# Autodesk Inventor assembly: CKK_145_NN_1_1800_mm_MF01_03_34_309_033
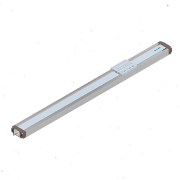
[picture p0: Inventor's stored thumbnail of the model, 180x180]
Saved by Autodesk Inventor 2021 (Build 250183000, 183)
## iProperties
Created: 2021-03-29
Part Number: CKK_145_NN_1_1800_mm_MF01_03_34_309_033
Document SubType Name: Assembly
Designer: Work
Sending System: CREO PARAMETRIC BY PTC INC, 2020044
Preprocessor: CREO PARAMETRIC BY PTC INC, 2020044
Title: R036050000_1800_ASM
Author: ac91sw
Revision Number: 1LAST_VERSION
## Documents named in this file (8)
- C:\Users\Work\OneDrive - Brookhaven National Laboratory\Daniels, William intern HPR station\Actuator\CKK_145_NN_1_1800_mm_MF01_03_34_309_033.iam
- C:\Users\Work\OneDrive - Brookhaven National Laboratory\Daniels, William intern HPR station\Actuator\R036050000_1800_SPDL.ipt
- C:\Users\Work\OneDrive - Brookhaven National Laboratory\Daniels, William intern HPR station\Actuator\R036050000_1800_HK.ipt
- C:\Users\Work\OneDrive - Brookhaven National Laboratory\Daniels, William intern HPR station\Actuator\R037250006_Z.ipt
- C:\Users\Work\OneDrive - Brookhaven National Laboratory\Daniels, William intern HPR station\Actuator\R037250005_Z.ipt
- C:\Users\Work\OneDrive - Brookhaven National Laboratory\Daniels, William intern HPR station\Actuator\R037550010_Z.ipt
- C:\Users\Work\OneDrive - Brookhaven National Laboratory\Daniels, William intern HPR station\Actuator\R037350043_Z.ipt
- C:\Users\Work\OneDrive - Brookhaven National Laboratory\Daniels, William intern HPR station\Actuator\R036050000_1800_ABD.ipt
## Components (8 placed, 8 different names)
1. 13 — Cylindrical:1
2. 14 — Rigid:2
3. 15 — Rigid:1, Rigid:2
4. 16 — Rigid:3
5. 17 — Rotational:1, Rotational:2
6. 18 — Rotational:1
7. 19 — Rotational:2, Cylindrical:1
8. 20 — Rigid:1, Rigid:3
## Relationships (6: WeldJoint 3, RevoluteJoint 2, CylindricalJoint 1)
- Rigid:1 [WeldJoint]: 15 ↔ 20
- Rigid:2 [WeldJoint] (1.4 mm): 14 ↔ 15
- Rigid:3 [WeldJoint]: 16 ↔ 20
- Rotational:1 [RevoluteJoint]: 17 ↔ 18
- Rotational:2 [RevoluteJoint]: 17 ↔ 19
- Cylindrical:1: 13 ↔ 19
